# Autodesk Inventor assembly: Shooter Assembly
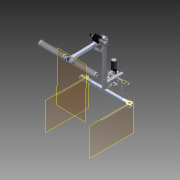
[picture p0: Inventor's stored thumbnail of the model, 180x180]
Saved by Autodesk Inventor 2014 SP1 (Build 180222100, 222)
## iProperties
Created: 2014-01-05
Part Number: Shooter Assembly
Document SubType Name: Assembly
Designer: Andrew Toennies
Mass: 7781.82 g
Surface Area: 22307.5 cm^2
Volume: 3128.72 cm^3
Density: 2.48722 g/cm^3
Author: Andrew Toennies
## Documents named in this file (27)
- C:\Users\Arpan\Documents\GitHub\2014buildCAD\Shooter\Shooter Assembly.iam
- C:\Users\Arpan\Documents\GitHub\2014buildCAD\Shooter\Vex Pro 1x1 rectangular tubing 12 in length.ipt
- C:\Users\Arpan\Documents\GitHub\2014buildCAD\Shooter\Vex Pro End Bearing Mount.ipt
- C:\Users\Arpan\Documents\GitHub\2014buildCAD\Shooter\Vex Pro 1x1 rectangular tubing 27 in length.ipt
- C:\Users\Arpan\Documents\GitHub\2014buildCAD\Shooter\Vex Pro 1x1 rectangular tubing 24 in length.ipt
- C:\Users\Arpan\Documents\GitHub\2014buildCAD\Shooter\Vex Pro Corner Gusset.ipt
- C:\Users\Arpan\Documents\GitHub\2014buildCAD\Shooter\Bearing ID 0.500 Hex OD 1.125.ipt
- C:\Users\Arpan\Documents\GitHub\2014buildCAD\Shooter\Spacer.ipt
- C:\Users\Arpan\Documents\GitHub\2014buildCAD\Shooter\Bearing ID 0.375 OD 1.125.ipt
- C:\Users\Arpan\Documents\GitHub\2014buildCAD\Shooter\Axle 0.375 3 in length.ipt
- C:\Users\Arpan\Documents\GitHub\2014buildCAD\Shooter\Axle 0.500 Hex 3 in length.ipt
- C:\Users\Arpan\Documents\GitHub\2014buildCAD\Shooter\Worm-Drive-Gearbox-16to1.iam
- C:\Users\Arpan\Documents\GitHub\2014buildCAD\Shooter\Vex Pro 32 tooth 15 mm timing belt pulley.ipt
- C:\Users\Arpan\Documents\GitHub\2014buildCAD\Shooter\Foot Bracket Mount (McMaster Part #6498K710).ipt
- C:\Users\Arpan\Documents\GitHub\2014buildCAD\Shooter\Rod End (McMaster Part #6498K592).ipt
- C:\Users\Arpan\Documents\GitHub\2014buildCAD\Shooter\Spacer2.ipt
- C:\Users\Arpan\Documents\GitHub\2014buildCAD\Shooter\Bracket.ipt
- C:\Users\Arpan\Documents\GitHub\2014buildCAD\Shooter\Axle 0.190 in 3 in length.ipt
- C:\Users\Arpan\Documents\GitHub\2014buildCAD\Shooter\6498K602 Pneumatic Cylinder Assembly.iam
- C:\Users\Arpan\Documents\GitHub\2014buildCAD\Shooter\mcmaster carr 32 tooth pulley.ipt
- C:\Users\Arpan\Documents\GitHub\2014buildCAD\Shooter\Vex Pro 1x1 rectangular tubing 4 in length.ipt
- C:\Users\Arpan\Documents\GitHub\2014buildCAD\Shooter\Vex Pro VersaFrame 90 Degree.ipt
- C:\Users\Arpan\Documents\GitHub\2014buildCAD\Shooter\Vex Pro Side Bearing Gusset.ipt
- C:\Users\Arpan\Documents\GitHub\2014buildCAD\Steel Plate (0.0625).ipt
- C:\Users\Arpan\Documents\GitHub\2014buildCAD\Collector\Drive Roller Assembly.iam
- C:\Users\Arpan\Documents\GitHub\2014buildCAD\Shooter\Vex Pro 1x1 rectangular tubing 7 in length.ipt
- C:\Users\Arpan\Documents\GitHub\2014buildCAD\Collector\12 inch pipe.ipt
## Components (48 placed, 26 different names)
1. Vex Pro Corner Gusset:1 — Insert:9, Insert:10, Flush:60, Flush:61
2. Vex Pro Corner Gusset:2 — Insert:11, Insert:12, Mate:261, Mate:262
3. Vex Pro End Bearing Mount:3 — Insert:35, Insert:47, Insert:48
4. Vex Pro End Bearing Mount:4 — Insert:36, Insert:49, Insert:50
5. Spacer:1 — Insert:47, Insert:48, Mate:65, Flush:24
6. Spacer:2 — Insert:49, Insert:50, Flush:22, Flush:23, Mate:64
7. Bearing ID 0.375 OD 1.125:1 — Insert:35, Mate:9
8. Bearing ID 0.375 OD 1.125:2 — Insert:36, Mate:66
9. Axle 0.375 3 in length:1 — Mate:9, Flush:9, Mate:66, Mate:269
10. Axle 0.500 Hex 3 in length:1 — Mate:47, Mate:48, Mate:210, Mate:211, Flush:59, Mate:250, Mate:251, Mate:258, Mate:259
11. Worm-Drive-Gearbox-16to1:1 [sub-assembly] — Mate:49, Mate:50, Mate:170, Mate:196, Mate:249
12. Vex Pro 32 tooth 15 mm timing belt pulley:1 — Mate:47, Mate:48, Flush:40, Rotation:1
13. Foot Bracket Mount (McMaster Part #6498K710):1 — Mate:71, Mate:72, Mate:73, Mate:99, Mate:100
14. Rod End (McMaster Part #6498K592):1 — Mate:102, Mate:103, Mate:194
15. Spacer2:1 — Mate:71, Mate:72, Mate:73, Mate:84, Mate:229
16. Bracket:1 — Mate:96, Flush:25, Mate:272, Mate:275, Mate:276
17. Bracket:2 — Mate:97, Mate:270, Mate:271, Mate:273, Mate:274
18. Axle 0.190 in 3 in length:1 — Mate:96, Mate:97, Flush:25, Mate:103
19. 6498K602 Pneumatic Cylinder Assembly:1 [sub-assembly] — Mate:99, Mate:100, Mate:102, Mate:194
20. mcmaster carr 32 tooth pulley:1 — Mate:170, Flush:40, Rotation:1, Mate:249, Flush:85
21. Bearing ID 0.500 Hex OD 1.125:4 — Flush:57, Mate:210, Flush:59, Insert:68
22. Bearing ID 0.500 Hex OD 1.125:3 — Insert:67
23. Bearing ID 0.500 Hex OD 1.125:7 — Flush:57, Mate:211, Insert:65, Flush:86
24. Vex Pro Corner Gusset:9 — Flush:60, Flush:61, Flush:64, Flush:65, Mate:218, Flush:66, Flush:67
25. Vex Pro Corner Gusset:10 — Flush:64, Flush:65, Mate:219, Mate:262
26. Vex Pro Side Bearing Gusset:1 — Mate:232, Mate:233, Mate:234, Insert:68
27. Vex Pro Side Bearing Gusset:2 — Mate:235, Mate:236, Mate:237, Insert:65
28. Vex Pro Side Bearing Gusset:3 — Mate:238, Mate:239, Mate:240, Insert:70
29. Vex Pro Side Bearing Gusset:4 — Mate:241, Mate:242, Mate:243, Insert:67
30. Vex Pro VersaFrame 90 Degree:1 — Mate:252, Mate:253, Mate:254
31. Vex Pro VersaFrame 90 Degree:2 — Mate:255, Mate:256, Mate:257
32. Vex Pro 32 tooth 15 mm timing belt pulley:2 — Mate:258, Mate:259, Flush:85
33. Bearing ID 0.500 Hex OD 1.125:8 — Insert:70, Flush:86
34. Steel Plate (0.0625):1 — Mate:263, Mate:264, Mate:265
35. Steel Plate (0.0625):2 — Mate:266, Mate:267, Mate:268
36. Drive Roller Assembly:1 [sub-assembly] — Mate:269, Mate:270, Mate:273, Mate:274, Mate:275, Mate:276
37. Vex Pro 1x1 rectangular tubing 7 in length:1 — Mate:277, Flush:87, Flush:88, Flush:89, Mate:287, Mate:288, Mate:289, Mate:290, Mate:291
38. Vex Pro 1x1 rectangular tubing 7 in length:2 — Mate:278, Flush:89, Flush:90, Mate:284, Mate:292, Mate:304, Mate:305
39. Vex Pro End Bearing Mount:5 — Mate:289, Mate:290, Mate:291
40. Vex Pro End Bearing Mount:6 — Mate:287, Mate:288, Mate:299
41. Vex Pro End Bearing Mount:7 — Mate:284, Mate:303, Flush:91, Mate:304, Mate:305
42. Vex Pro End Bearing Mount:8 — Mate:292, Mate:300, Mate:303, Flush:91
43. 12 inch pipe:1 — Mate:300
44. 12 inch pipe:2 — Mate:299
45. Vex Pro 1x1 rectangular tubing 4 in length:1 — Mate:218, Flush:66, Flush:67, Mate:219, Mate:235, Mate:236, Mate:237, Mate:238, Mate:239, Mate:240, Angle:1
46. Vex Pro 1x1 rectangular tubing 12 in length:1 — Insert:9, Insert:10, Insert:11, Insert:12, Mate:49, Mate:50, Mate:196, Mate:232, Mate:233, Mate:234, Mate:241, Mate:242, Mate:243
47. Vex Pro 1x1 rectangular tubing 27 in length:1 — Flush:2, Mate:2, Mate:250, Mate:251, Mate:254, Mate:261, Mate:263, Mate:264, Mate:265, Mate:266, Mate:267, Mate:268, Angle:1
48. Vex Pro 1x1 rectangular tubing 24 in length:1 — Flush:2, Mate:2, Flush:9, Flush:22, Flush:23, Mate:64, Mate:65, Flush:24, Mate:84, Mate:229, Flush:79, Mate:252, Mate:253, Mate:255, Mate:256, Mate:257, Mate:271, Mate:272, Mate:277, Flush:87, Flush:88, Mate:278, Flush:90
## Relationships (119: Mate 80, Flush 23, Insert 14, RelateRotation 1, Angle 1)
- Flush:2: Vex Pro 1x1 rectangular tubing 27 in length:1 ↔ Vex Pro 1x1 rectangular tubing 24 in length:1
- Mate:2: Vex Pro 1x1 rectangular tubing 27 in length:1 ↔ Vex Pro 1x1 rectangular tubing 24 in length:1
- Insert:9: Vex Pro Corner Gusset:1 ↔ Vex Pro 1x1 rectangular tubing 12 in length:1
- Insert:10: Vex Pro Corner Gusset:1 ↔ Vex Pro 1x1 rectangular tubing 12 in length:1
- Insert:11: Vex Pro Corner Gusset:2 ↔ Vex Pro 1x1 rectangular tubing 12 in length:1
- Insert:12: Vex Pro Corner Gusset:2 ↔ Vex Pro 1x1 rectangular tubing 12 in length:1
- Insert:35: Vex Pro End Bearing Mount:3 ↔ Bearing ID 0.375 OD 1.125:1
- Insert:36: Vex Pro End Bearing Mount:4 ↔ Bearing ID 0.375 OD 1.125:2
- Mate:9: Bearing ID 0.375 OD 1.125:1 ↔ Axle 0.375 3 in length:1
- Flush:9 (-25.4 mm): Axle 0.375 3 in length:1 ↔ Vex Pro 1x1 rectangular tubing 24 in length:1
- Mate:47: Axle 0.500 Hex 3 in length:1 ↔ Vex Pro 32 tooth 15 mm timing belt pulley:1
- Mate:48: Axle 0.500 Hex 3 in length:1 ↔ Vex Pro 32 tooth 15 mm timing belt pulley:1
- Mate:49: Worm-Drive-Gearbox-16to1:1 ↔ Vex Pro 1x1 rectangular tubing 12 in length:1
- Mate:50: Worm-Drive-Gearbox-16to1:1 ↔ Vex Pro 1x1 rectangular tubing 12 in length:1
- Insert:47: Vex Pro End Bearing Mount:3 ↔ Spacer:1
- Insert:48: Vex Pro End Bearing Mount:3 ↔ Spacer:1
- Insert:49: Vex Pro End Bearing Mount:4 ↔ Spacer:2
- Insert:50: Vex Pro End Bearing Mount:4 ↔ Spacer:2
- Flush:22: Spacer:2 ↔ Vex Pro 1x1 rectangular tubing 24 in length:1
- Flush:23: Spacer:2 ↔ Vex Pro 1x1 rectangular tubing 24 in length:1
- Mate:64: Spacer:2 ↔ Vex Pro 1x1 rectangular tubing 24 in length:1
- Mate:65: Spacer:1 ↔ Vex Pro 1x1 rectangular tubing 24 in length:1
- Flush:24: Spacer:1 ↔ Vex Pro 1x1 rectangular tubing 24 in length:1
- Mate:66: Bearing ID 0.375 OD 1.125:2 ↔ Axle 0.375 3 in length:1
- Mate:71: Foot Bracket Mount (McMaster Part #6498K710):1 ↔ Spacer2:1
- Mate:72: Foot Bracket Mount (McMaster Part #6498K710):1 ↔ Spacer2:1
- Mate:73: Foot Bracket Mount (McMaster Part #6498K710):1 ↔ Spacer2:1
- Mate:84: Spacer2:1 ↔ Vex Pro 1x1 rectangular tubing 24 in length:1
- Mate:96: Bracket:1 ↔ Axle 0.190 in 3 in length:1
- Mate:97: Bracket:2 ↔ Axle 0.190 in 3 in length:1
- Flush:25 (-11.1125 mm): Bracket:1 ↔ Axle 0.190 in 3 in length:1
- Mate:99: Foot Bracket Mount (McMaster Part #6498K710):1 ↔ 6498K602 Pneumatic Cylinder Assembly:1
- Mate:100: Foot Bracket Mount (McMaster Part #6498K710):1 ↔ 6498K602 Pneumatic Cylinder Assembly:1
- Mate:102: Rod End (McMaster Part #6498K592):1 ↔ 6498K602 Pneumatic Cylinder Assembly:1
- Mate:103: Rod End (McMaster Part #6498K592):1 ↔ Axle 0.190 in 3 in length:1
- Mate:170: Worm-Drive-Gearbox-16to1:1 ↔ mcmaster carr 32 tooth pulley:1
- Flush:40: Vex Pro 32 tooth 15 mm timing belt pulley:1 ↔ mcmaster carr 32 tooth pulley:1
- Rotation:1 [RelateRotation] (1 ul): Vex Pro 32 tooth 15 mm timing belt pulley:1 ↔ mcmaster carr 32 tooth pulley:1
- Mate:194 (-12.7 mm): Rod End (McMaster Part #6498K592):1 ↔ 6498K602 Pneumatic Cylinder Assembly:1
- Mate:196: Worm-Drive-Gearbox-16to1:1 ↔ Vex Pro 1x1 rectangular tubing 12 in length:1
- Flush:57: Bearing ID 0.500 Hex OD 1.125:4 ↔ Bearing ID 0.500 Hex OD 1.125:7
- Mate:210: Axle 0.500 Hex 3 in length:1 ↔ Bearing ID 0.500 Hex OD 1.125:4
- Mate:211: Axle 0.500 Hex 3 in length:1 ↔ Bearing ID 0.500 Hex OD 1.125:7
- Flush:59 (12.7 mm): Axle 0.500 Hex 3 in length:1 ↔ Bearing ID 0.500 Hex OD 1.125:4
- Flush:60: Vex Pro Corner Gusset:1 ↔ Vex Pro Corner Gusset:9
- Flush:61: Vex Pro Corner Gusset:1 ↔ Vex Pro Corner Gusset:9
- Flush:64: Vex Pro Corner Gusset:9 ↔ Vex Pro Corner Gusset:10
- Flush:65: Vex Pro Corner Gusset:9 ↔ Vex Pro Corner Gusset:10
- Mate:218: Vex Pro Corner Gusset:9 ↔ Vex Pro 1x1 rectangular tubing 4 in length:1
- Flush:66: Vex Pro Corner Gusset:9 ↔ Vex Pro 1x1 rectangular tubing 4 in length:1
- Flush:67: Vex Pro Corner Gusset:9 ↔ Vex Pro 1x1 rectangular tubing 4 in length:1
- Mate:219: Vex Pro Corner Gusset:10 ↔ Vex Pro 1x1 rectangular tubing 4 in length:1
- Mate:229: Spacer2:1 ↔ Vex Pro 1x1 rectangular tubing 24 in length:1
- Flush:79 (330.2 mm): Vex Pro 1x1 rectangular tubing 24 in length:1
- Mate:232: Vex Pro Side Bearing Gusset:1 ↔ Vex Pro 1x1 rectangular tubing 12 in length:1
- Mate:233: Vex Pro Side Bearing Gusset:1 ↔ Vex Pro 1x1 rectangular tubing 12 in length:1
- Mate:234: Vex Pro Side Bearing Gusset:1 ↔ Vex Pro 1x1 rectangular tubing 12 in length:1
- Mate:235: Vex Pro Side Bearing Gusset:2 ↔ Vex Pro 1x1 rectangular tubing 4 in length:1
- Mate:236: Vex Pro Side Bearing Gusset:2 ↔ Vex Pro 1x1 rectangular tubing 4 in length:1
- Mate:237: Vex Pro Side Bearing Gusset:2 ↔ Vex Pro 1x1 rectangular tubing 4 in length:1
- Mate:238: Vex Pro Side Bearing Gusset:3 ↔ Vex Pro 1x1 rectangular tubing 4 in length:1
- Mate:239: Vex Pro Side Bearing Gusset:3 ↔ Vex Pro 1x1 rectangular tubing 4 in length:1
- Mate:240: Vex Pro Side Bearing Gusset:3 ↔ Vex Pro 1x1 rectangular tubing 4 in length:1
- Mate:241: Vex Pro Side Bearing Gusset:4 ↔ Vex Pro 1x1 rectangular tubing 12 in length:1
- Mate:242: Vex Pro Side Bearing Gusset:4 ↔ Vex Pro 1x1 rectangular tubing 12 in length:1
- Mate:243: Vex Pro Side Bearing Gusset:4 ↔ Vex Pro 1x1 rectangular tubing 12 in length:1
- Insert:65: Bearing ID 0.500 Hex OD 1.125:7 ↔ Vex Pro Side Bearing Gusset:2
- Insert:67: Bearing ID 0.500 Hex OD 1.125:3 ↔ Vex Pro Side Bearing Gusset:4
- Insert:68: Bearing ID 0.500 Hex OD 1.125:4 ↔ Vex Pro Side Bearing Gusset:1
- Mate:249 (12.7 mm): Worm-Drive-Gearbox-16to1:1 ↔ mcmaster carr 32 tooth pulley:1
- Mate:250: Axle 0.500 Hex 3 in length:1 ↔ Vex Pro 1x1 rectangular tubing 27 in length:1
- Mate:251: Axle 0.500 Hex 3 in length:1 ↔ Vex Pro 1x1 rectangular tubing 27 in length:1
- Mate:252: Vex Pro VersaFrame 90 Degree:1 ↔ Vex Pro 1x1 rectangular tubing 24 in length:1
- Mate:253: Vex Pro VersaFrame 90 Degree:1 ↔ Vex Pro 1x1 rectangular tubing 24 in length:1
- Mate:254: Vex Pro VersaFrame 90 Degree:1 ↔ Vex Pro 1x1 rectangular tubing 27 in length:1
- Mate:255: Vex Pro VersaFrame 90 Degree:2 ↔ Vex Pro 1x1 rectangular tubing 24 in length:1
- Mate:256: Vex Pro VersaFrame 90 Degree:2 ↔ Vex Pro 1x1 rectangular tubing 24 in length:1
- Mate:257: Vex Pro VersaFrame 90 Degree:2 ↔ Vex Pro 1x1 rectangular tubing 24 in length:1
- Mate:258: Axle 0.500 Hex 3 in length:1 ↔ Vex Pro 32 tooth 15 mm timing belt pulley:2
- Mate:259: Axle 0.500 Hex 3 in length:1 ↔ Vex Pro 32 tooth 15 mm timing belt pulley:2
- Flush:85: mcmaster carr 32 tooth pulley:1 ↔ Vex Pro 32 tooth 15 mm timing belt pulley:2
- Insert:70: Vex Pro Side Bearing Gusset:3 ↔ Bearing ID 0.500 Hex OD 1.125:8
- Flush:86: Bearing ID 0.500 Hex OD 1.125:7 ↔ Bearing ID 0.500 Hex OD 1.125:8
- Mate:261: Vex Pro Corner Gusset:2 ↔ Vex Pro 1x1 rectangular tubing 27 in length:1
- Mate:262 (31.75 mm): Vex Pro Corner Gusset:2 ↔ Vex Pro Corner Gusset:10
- Mate:263: Steel Plate (0.0625):1 ↔ Vex Pro 1x1 rectangular tubing 27 in length:1
- Mate:264: Steel Plate (0.0625):1 ↔ Vex Pro 1x1 rectangular tubing 27 in length:1
- Mate:265: Steel Plate (0.0625):1 ↔ Vex Pro 1x1 rectangular tubing 27 in length:1
- Mate:266: Steel Plate (0.0625):2 ↔ Vex Pro 1x1 rectangular tubing 27 in length:1
- Mate:267: Steel Plate (0.0625):2 ↔ Vex Pro 1x1 rectangular tubing 27 in length:1
- Mate:268: Steel Plate (0.0625):2 ↔ Vex Pro 1x1 rectangular tubing 27 in length:1
- Mate:269: Axle 0.375 3 in length:1 ↔ Drive Roller Assembly:1
- Mate:270: Bracket:2 ↔ Drive Roller Assembly:1
- Mate:271: Bracket:2 ↔ Vex Pro 1x1 rectangular tubing 24 in length:1
- Mate:272: Bracket:1 ↔ Vex Pro 1x1 rectangular tubing 24 in length:1
- Mate:273: Bracket:2 ↔ Drive Roller Assembly:1
- Mate:274: Bracket:2 ↔ Drive Roller Assembly:1
- Mate:275: Bracket:1 ↔ Drive Roller Assembly:1
- Mate:276: Bracket:1 ↔ Drive Roller Assembly:1
- Angle:1 (0 deg): Vex Pro 1x1 rectangular tubing 4 in length:1 ↔ Vex Pro 1x1 rectangular tubing 27 in length:1
- Mate:277: Vex Pro 1x1 rectangular tubing 7 in length:1 ↔ Vex Pro 1x1 rectangular tubing 24 in length:1
- Flush:87: Vex Pro 1x1 rectangular tubing 7 in length:1 ↔ Vex Pro 1x1 rectangular tubing 24 in length:1
- Flush:88: Vex Pro 1x1 rectangular tubing 7 in length:1 ↔ Vex Pro 1x1 rectangular tubing 24 in length:1
- Mate:278: Vex Pro 1x1 rectangular tubing 7 in length:2 ↔ Vex Pro 1x1 rectangular tubing 24 in length:1
- Flush:89: Vex Pro 1x1 rectangular tubing 7 in length:1 ↔ Vex Pro 1x1 rectangular tubing 7 in length:2
- Flush:90: Vex Pro 1x1 rectangular tubing 7 in length:2 ↔ Vex Pro 1x1 rectangular tubing 24 in length:1
- Mate:284: Vex Pro 1x1 rectangular tubing 7 in length:2 ↔ Vex Pro End Bearing Mount:7
- Mate:287: Vex Pro 1x1 rectangular tubing 7 in length:1 ↔ Vex Pro End Bearing Mount:6
- Mate:288: Vex Pro 1x1 rectangular tubing 7 in length:1 ↔ Vex Pro End Bearing Mount:6
- Mate:289: Vex Pro 1x1 rectangular tubing 7 in length:1 ↔ Vex Pro End Bearing Mount:5
- Mate:290: Vex Pro 1x1 rectangular tubing 7 in length:1 ↔ Vex Pro End Bearing Mount:5
- Mate:291: Vex Pro 1x1 rectangular tubing 7 in length:1 ↔ Vex Pro End Bearing Mount:5
- Mate:292: Vex Pro 1x1 rectangular tubing 7 in length:2 ↔ Vex Pro End Bearing Mount:8
- Mate:299: Vex Pro End Bearing Mount:6 ↔ 12 inch pipe:2
- Mate:300: Vex Pro End Bearing Mount:8 ↔ 12 inch pipe:1
- Mate:303: Vex Pro End Bearing Mount:7 ↔ Vex Pro End Bearing Mount:8
- Flush:91: Vex Pro End Bearing Mount:7 ↔ Vex Pro End Bearing Mount:8
- Mate:304: Vex Pro 1x1 rectangular tubing 7 in length:2 ↔ Vex Pro End Bearing Mount:7
- Mate:305: Vex Pro 1x1 rectangular tubing 7 in length:2 ↔ Vex Pro End Bearing Mount:7
